# Autodesk Inventor assembly: 1103 Robot - Base2
(part 2 of 2)
- Mate:349: Flat Bearing Block:15 ↔ Nut 8-32 Nylock:9
- Mate:350: Screw 8-32 x 0.500''-Silver:13 ↔ Nut 8-32 Nylock:9
- Mate:351: Screw 8-32 x 0.500''-Silver:14 ↔ Nut 8-32 Nylock:8
- Mate:352: Flat Bearing Block:13 ↔ Nut 8-32 Nylock:10
- Mate:353: Flat Bearing Block:13 ↔ Nut 8-32 Nylock:11
- Mate:354: Screw 8-32 x 0.500''-Silver:9 ↔ Nut 8-32 Nylock:11
- Mate:355: Screw 8-32 x 0.500''-Silver:10 ↔ Nut 8-32 Nylock:10
- Mate:356: Flat Bearing Block:3 ↔ Nut 8-32 Nylock:12
- Mate:357: Flat Bearing Block:3 ↔ Nut 8-32 Nylock:13
- Mate:358: Flat Bearing Block:4 ↔ Nut 8-32 Nylock:14
- Mate:359: Flat Bearing Block:4 ↔ Nut 8-32 Nylock:15
- Mate:360: Flat Bearing Block:5 ↔ Nut 8-32 Nylock:17
- Mate:361: Flat Bearing Block:5 ↔ Nut 8-32 Nylock:16
- Mate:362: Screw 8-32 x 0.500''-Silver:6 ↔ Nut 8-32 Nylock:17
- Mate:363: Screw 8-32 x 0.500''-Silver:5 ↔ Nut 8-32 Nylock:16
- Mate:364: Screw 8-32 x 0.500''-Silver:4 ↔ Nut 8-32 Nylock:14
- Mate:365: Screw 8-32 x 0.500''-Silver:3 ↔ Nut 8-32 Nylock:15
- Mate:366: Screw 8-32 x 0.500''-Silver:1 ↔ Nut 8-32 Nylock:12
- Mate:367: Screw 8-32 x 0.500''-Silver:2 ↔ Nut 8-32 Nylock:13
- Mate:368: 2 x 6:1 ↔ Screw 8-32 x 0.250''-Silver:1
- Mate:369: 2 x 6:1 ↔ Screw 8-32 x 0.250''-Silver:2
- Mate:370: 2 x 6:2 ↔ Screw 8-32 x 0.250''-Silver:4
- Mate:371: 2 x 6:2 ↔ Screw 8-32 x 0.250''-Silver:3
- Mate:372: Standoff 0.50'':5 ↔ Screw 8-32 x 0.250''-Silver:1
- Mate:373: Standoff 0.50'':8 ↔ Screw 8-32 x 0.250''-Silver:2
- Mate:374: Standoff 0.50'':6 ↔ Screw 8-32 x 0.250''-Silver:4
- Mate:375: Standoff 0.50'':7 ↔ Screw 8-32 x 0.250''-Silver:3
- Mate:376: 2 x 6:4 ↔ Screw 8-32 x 0.250''-Silver:8
- Mate:377: 2 x 6:4 ↔ Screw 8-32 x 0.250''-Silver:7
- Mate:378: 2 x 6:3 ↔ Screw 8-32 x 0.250''-Silver:6
- Mate:379: 2 x 6:3 ↔ Screw 8-32 x 0.250''-Silver:5
- Mate:380: Standoff 0.50'':3 ↔ Screw 8-32 x 0.250''-Silver:6
- Mate:381: Standoff 0.50'':1 ↔ Screw 8-32 x 0.250''-Silver:5
- Mate:382: Standoff 0.50'':4 ↔ Screw 8-32 x 0.250''-Silver:7
- Mate:383: Standoff 0.50'':2 ↔ Screw 8-32 x 0.250''-Silver:8
- Mate:384: 4 Slotted Angle:1 ↔ Screw 8-32 x 0.250''-Silver:9
- Mate:385: 4 Slotted Angle:1 ↔ Screw 8-32 x 0.250''-Silver:10
- Mate:386: Standoff 0.50'':9 ↔ Screw 8-32 x 0.250''-Silver:9
- Mate:387: Standoff 0.50'':10 ↔ Screw 8-32 x 0.250''-Silver:10
- Mate:388: 4 Slotted Angle:2 ↔ Screw 8-32 x 0.250''-Silver:11
- Mate:389: 4 Slotted Angle:2 ↔ Screw 8-32 x 0.250''-Silver:12
- Mate:390: Standoff 0.50'':11 ↔ Screw 8-32 x 0.250''-Silver:12
- Mate:391: Standoff 0.50'':12 ↔ Screw 8-32 x 0.250''-Silver:11
- [Mate]: 4 x 6 cut:1 ↔ Screw 8-32 x 0.375''-Silver:1
- [Mate]: 4 x 6 cut:1 ↔ Screw 8-32 x 0.375''-Silver:2
- [Tangent] (0.2286 mm): 4 x 6 cut:1 ↔ Screw 8-32 x 0.375''-Silver:1
- [Tangent] (0.2286 mm): 4 x 6 cut:1 ↔ Screw 8-32 x 0.375''-Silver:1
- [Tangent] (0.2286 mm): 4 x 6 cut:1 ↔ Screw 8-32 x 0.375''-Silver:2
- [Tangent] (0.2286 mm): 4 x 6 cut:1 ↔ Screw 8-32 x 0.375''-Silver:2
- [Mate]: Ultrasonic Range Finder (Sensor):1 ↔ Nut 8-32 Keps:2
- [Mate]: Ultrasonic Range Finder (Sensor):1 ↔ Nut 8-32 Keps:1
- [Mate]: Screw 8-32 x 0.375''-Silver:1 ↔ Nut 8-32 Keps:1
- [Mate]: Screw 8-32 x 0.375''-Silver:2 ↔ Nut 8-32 Keps:2
- [Tangent] (0.2286 mm): 4 x 6 cut:2 ↔ Screw 8-32 x 0.375''-Silver:3
- [Tangent] (0.2286 mm): 4 x 6 cut:2 ↔ Screw 8-32 x 0.375''-Silver:3
- [Mate]: 4 x 6 cut:2 ↔ Screw 8-32 x 0.375''-Silver:3
- [Tangent] (0.2286 mm): 4 x 6 cut:2 ↔ Screw 8-32 x 0.375''-Silver:4
- [Tangent] (0.2286 mm): 4 x 6 cut:2 ↔ Screw 8-32 x 0.375''-Silver:4
- [Mate]: 4 x 6 cut:2 ↔ Screw 8-32 x 0.375''-Silver:4
- [Mate]: Ultrasonic Range Finder (Sensor):2 ↔ Nut 8-32 Keps:3
- [Mate]: Ultrasonic Range Finder (Sensor):2 ↔ Nut 8-32 Keps:4
- [Mate]: Nut 8-32 Keps:4 ↔ Screw 8-32 x 0.375''-Silver:3
- [Mate]: Nut 8-32 Keps:3 ↔ Screw 8-32 x 0.375''-Silver:4
- Mate:406: 4 x 6 cut:2 ↔ Screw 8-32 x 0.750''-Silver:1
- Mate:407: 4 x 6 cut:2 ↔ Screw 8-32 x 0.750''-Silver:2
- Mate:408: Spacer (Nylon), 0.375'':3 ↔ Screw 8-32 x 0.750''-Silver:1
- Mate:409: Spacer (Nylon), 0.375'':4 ↔ Screw 8-32 x 0.750''-Silver:2
- Mate:410: 4 Slotted Angle:2 ↔ Nut 8-32 Nylock:18
- Mate:411: 4 Slotted Angle:2 ↔ Nut 8-32 Nylock:19
- Mate:412: Screw 8-32 x 0.750''-Silver:2 ↔ Nut 8-32 Nylock:19
- Mate:413: Screw 8-32 x 0.750''-Silver:1 ↔ Nut 8-32 Nylock:18
- Mate:414: 4 x 6 cut:1 ↔ Screw 8-32 x 0.750''-Silver:3
- Mate:415: 4 x 6 cut:1 ↔ Screw 8-32 x 0.750''-Silver:4
- Mate:416: Spacer (Nylon), 0.375'':1 ↔ Screw 8-32 x 0.750''-Silver:3
- Mate:417: Spacer (Nylon), 0.375'':2 ↔ Screw 8-32 x 0.750''-Silver:4
- Mate:418: 4 Slotted Angle:1 ↔ Nut 8-32 Nylock:20
- Mate:419: 4 Slotted Angle:1 ↔ Nut 8-32 Nylock:21
- Mate:420: Screw 8-32 x 0.750''-Silver:4 ↔ Nut 8-32 Nylock:21
- Mate:421: Screw 8-32 x 0.750''-Silver:3 ↔ Nut 8-32 Nylock:20
- Tangent:171 (0.2311 mm): 1103 Custom Chassis:1 ↔ .375'' Screw & Nylock Nut:1
- Tangent:172 (0.2286 mm): 1103 Custom Chassis:1 ↔ .375'' Screw & Nylock Nut:1
- Mate:422: 5 x 24:1 ↔ .375'' Screw & Nylock Nut:1
- Mate:423: 1103 Custom Chassis:1 ↔ .375'' Screw & Nylock Nut:3
- Tangent:173 (0.2286 mm): 1103 Custom Chassis:1 ↔ .375'' Screw & Nylock Nut:3
- Tangent:174 (0.2286 mm): 1103 Custom Chassis:1 ↔ .375'' Screw & Nylock Nut:3
- Mate:424: 1103 Custom Chassis:1 ↔ .375'' Screw & Nylock Nut:4
- Mate:425: 1103 Custom Chassis:1 ↔ .375'' Screw & Nylock Nut:2
- Tangent:175 (0.2286 mm): 1103 Custom Chassis:1 ↔ .375'' Screw & Nylock Nut:2
- Tangent:176 (0.2286 mm): 1103 Custom Chassis:1 ↔ .375'' Screw & Nylock Nut:2
- Tangent:177: 1103 Custom Chassis:1 ↔ .375'' Screw & Nylock Nut:4
- Mate:426: 1103 Custom Chassis:1 ↔ .375'' Screw & Nylock Nut:5
- Mate:427: 1103 Custom Chassis:1 ↔ .375'' Screw & Nylock Nut:6
- Tangent:178 (0.2286 mm): 1103 Custom Chassis:1 ↔ .375'' Screw & Nylock Nut:5
- Tangent:179 (0.2286 mm): 1103 Custom Chassis:1 ↔ .375'' Screw & Nylock Nut:5
- Tangent:180 (0.2286 mm): 1103 Custom Chassis:1 ↔ .375'' Screw & Nylock Nut:6
- Tangent:181 (0.2286 mm): 1103 Custom Chassis:1 ↔ .375'' Screw & Nylock Nut:6
- Mate:428: 1103 Custom Chassis:1 ↔ .375'' Screw & Nylock Nut:7
- Mate:429: 1103 Custom Chassis:1 ↔ .375'' Screw & Nylock Nut:8
- Tangent:182 (0.2286 mm): 1103 Custom Chassis:1 ↔ .375'' Screw & Nylock Nut:8
- Tangent:183 (0.2286 mm): 1103 Custom Chassis:1 ↔ .375'' Screw & Nylock Nut:8
- Tangent:184 (0.2286 mm): 1103 Custom Chassis:1 ↔ .375'' Screw & Nylock Nut:7
- Tangent:185 (0.2286 mm): 1103 Custom Chassis:1 ↔ .375'' Screw & Nylock Nut:7
- Mate:430: 5 x 25 Custom:1 ↔ .375'' Screw & Nylock Nut:9
- Tangent:186 (0.2286 mm): 5 x 24:1 ↔ .375'' Screw & Nylock Nut:9
- Tangent:187 (0.2286 mm): 5 x 25 Custom:1 ↔ .375'' Screw & Nylock Nut:9
- Mate:431: 5 x 25 Custom:1 ↔ .375'' Screw & Nylock Nut:10
- Tangent:188 (0.2286 mm): 5 x 25 Custom:1 ↔ .375'' Screw & Nylock Nut:10
- Tangent:189 (0.2286 mm): 5 x 25 Custom:1 ↔ .375'' Screw & Nylock Nut:10
- Mate:432: 5 x 24:1 ↔ .375'' Screw & Nylock Nut:11
- Tangent:190 (0.2286 mm): 5 x 24:1 ↔ .375'' Screw & Nylock Nut:11
- Tangent:191 (0.2286 mm): 5 x 24:1 ↔ .375'' Screw & Nylock Nut:11
- Mate:433: 5 x 24:2 ↔ .375'' Screw & Nylock Nut:12
- Tangent:192 (0.2286 mm): 5 x 24:2 ↔ .375'' Screw & Nylock Nut:12
- Tangent:193 (0.2286 mm): 5 x 24:2 ↔ .375'' Screw & Nylock Nut:12
- Mate:434 (3.175 mm): 2 x 25:1 ↔ VEX-HINGE-1 RevA_1:1
- Mate:435 (3.175 mm): 2 x 25:1 ↔ VEX-HINGE-1 RevA 4x:1
- Mate:436: VEX-HINGE-1 RevA 4x:1 ↔ VEX-HINGE-PIN 4x:1
- Mate:437: VEX-HINGE-1 RevA_1:1 ↔ VEX-HINGE-PIN_1:1
- Flush:60: VEX-HINGE-1 RevA_1:1 ↔ VEX-HINGE-PIN_1:1
- Flush:61: VEX-HINGE-1 RevA 4x:1 ↔ VEX-HINGE-PIN 4x:1
- Flush:62: 2 x 25:1 ↔ VEX-HINGE-1 RevA_1:1
- Flush:63: 2 x 25:1 ↔ VEX-HINGE-1 RevA_1:1
- Flush:64: 2 x 25:1 ↔ VEX-HINGE-1 RevA 4x:1
- Flush:65: 2 x 25:1 ↔ VEX-HINGE-1 RevA 4x:1
- Flush:66 (2.3114 mm): VEX-HINGE-1 RevA_1:1
- Mate:448: 2 x 25:1 ↔ .375'' Screw & Nylock Nut:18
- Mate:449: 2 x 25:1 ↔ .375'' Screw & Nylock Nut:19
- Tangent:199 (0.2286 mm): 2 x 25:1 ↔ .375'' Screw & Nylock Nut:18
- Tangent:200 (0.2286 mm): 2 x 25:1 ↔ .375'' Screw & Nylock Nut:18
- Tangent:201 (0.2286 mm): 2 x 25:1 ↔ .375'' Screw & Nylock Nut:19
- Tangent:202 (0.2286 mm): 2 x 25:1 ↔ .375'' Screw & Nylock Nut:19
- Mate:450: 2 x 25:1 ↔ .375'' Screw & Nylock Nut:20
- Mate:451: 2 x 25:1 ↔ .375'' Screw & Nylock Nut:21
- Tangent:203 (0.2286 mm): 2 x 25:1 ↔ .375'' Screw & Nylock Nut:20
- Tangent:204 (0.2286 mm): 2 x 25:1 ↔ .375'' Screw & Nylock Nut:20
- Tangent:205 (0.2286 mm): 2 x 25:1 ↔ .375'' Screw & Nylock Nut:21
- Tangent:206 (0.2286 mm): 2 x 25:1 ↔ .375'' Screw & Nylock Nut:21
- Mate:452: 5 x 24:1 ↔ 2 x 25:1
- Flush:67: 5 x 24:1 ↔ 2 x 25:1
- Tangent:207 (0.2286 mm): 1103 Custom Chassis:1 ↔ .375'' Screw & Nylock Nut:4
- Mate:453: 2 x 25:1 ↔ Spacer (Nylon), 0.125'':1
- Tangent:208: VEX-HINGE-1 RevA 4x:1 ↔ Spacer (Nylon), 0.125'':1
- Tangent:209: VEX-HINGE-1 RevA 4x:1 ↔ Spacer (Nylon), 0.125'':1
- Mate:454: Screw 8-32 x 0.500''-Silver:19 ↔ Spacer (Nylon), 0.125'':1
- Mate:455: VEX-HINGE-1 RevA 4x:1 ↔ Screw 8-32 x 0.500''-Silver:19
- Mate:456: 2 x 25:1 ↔ Spacer (Nylon), 0.125'':2
- Mate:457: 2 x 25:1 ↔ Spacer (Nylon), 0.125'':3
- Mate:458: 2 x 25:1 ↔ Spacer (Nylon), 0.125'':4
- Mate:459: 2 x 25:1 ↔ Spacer (Nylon), 0.125'':5
- Tangent:210: VEX-HINGE-1 RevA_1:1 ↔ Spacer (Nylon), 0.125'':5
- Tangent:211: VEX-HINGE-1 RevA_1:1 ↔ Spacer (Nylon), 0.125'':5
- Tangent:212 (-0.2286 mm): VEX-HINGE-1 RevA_1:1 ↔ Spacer (Nylon), 0.125'':4
- Tangent:213 (-0.2286 mm): VEX-HINGE-1 RevA_1:1 ↔ Spacer (Nylon), 0.125'':4
- Tangent:214 (-0.2286 mm): VEX-HINGE-1 RevA_1:1 ↔ Spacer (Nylon), 0.125'':3
- Tangent:215 (-0.2286 mm): VEX-HINGE-1 RevA_1:1 ↔ Spacer (Nylon), 0.125'':3
- Tangent:216 (-0.2286 mm): VEX-HINGE-1 RevA 4x:1 ↔ Spacer (Nylon), 0.125'':2
- Tangent:217 (-0.2286 mm): VEX-HINGE-1 RevA 4x:1 ↔ Spacer (Nylon), 0.125'':2
- Mate:460: Screw 8-32 x 0.500''-Silver:20 ↔ Spacer (Nylon), 0.125'':2
- Mate:461: Screw 8-32 x 0.500''-Silver:21 ↔ Spacer (Nylon), 0.125'':3
- Mate:462: Screw 8-32 x 0.500''-Silver:22 ↔ Spacer (Nylon), 0.125'':4
- Mate:463: Screw 8-32 x 0.500''-Silver:23 ↔ Spacer (Nylon), 0.125'':5
- Mate:464: VEX-HINGE-1 RevA_1:1 ↔ Screw 8-32 x 0.500''-Silver:23
- Mate:465: VEX-HINGE-1 RevA_1:1 ↔ Screw 8-32 x 0.500''-Silver:22
- Mate:466: VEX-HINGE-1 RevA_1:1 ↔ Screw 8-32 x 0.500''-Silver:21
- Mate:467: VEX-HINGE-1 RevA 4x:1 ↔ Screw 8-32 x 0.500''-Silver:20
- Mate:468: 2 x 25:1 ↔ Nut 8-32 Nylock:22
- Mate:469: 2 x 25:1 ↔ Nut 8-32 Nylock:23
- Mate:470: 2 x 25:1 ↔ Nut 8-32 Nylock:24
- Mate:471: 2 x 25:1 ↔ Nut 8-32 Nylock:25
- Mate:472: 2 x 25:1 ↔ Nut 8-32 Nylock:26
- Mate:473: Screw 8-32 x 0.500''-Silver:23 ↔ Nut 8-32 Nylock:22
- Mate:474: Screw 8-32 x 0.500''-Silver:22 ↔ Nut 8-32 Nylock:23
- Mate:475: Screw 8-32 x 0.500''-Silver:21 ↔ Nut 8-32 Nylock:24
- Mate:476: Screw 8-32 x 0.500''-Silver:20 ↔ Nut 8-32 Nylock:25
- Mate:477: Screw 8-32 x 0.500''-Silver:19 ↔ Nut 8-32 Nylock:26
- Mate:478: Flat Bearing Block:8 ↔ 2-Wire Motor 393-Without Wire:2
- Mate:479: Flat Bearing Block:8 ↔ Screw 6-32 x 0.500''-Silver:9
- Mate:480: 2-Wire Motor 393-Without Wire:2 ↔ Screw 6-32 x 0.500''-Silver:9
- Mate:481: 5 x 24:1 ↔ Screw 6-32 x 0.500''-Silver:9
- Mate:482: 5 x 24:1 ↔ Drivetrain Encoder:1
- Flush:68: 5 x 24:1 ↔ Drivetrain Encoder:1
- Mate:483: 5 x 25 Custom:1 ↔ Drivetrain Encoder:1
- Mate:484: Drivetrain Encoder:1 ↔ Bearing Block:5
- Mate:485: 5 x 24:1 ↔ Bearing Block:5
- Tangent:220 (0.1905 mm): 5 x 24:1 ↔ Bearing Block:5
- Mate:486: 5 x 24:2 ↔ Bearing Block:6
- Tangent:221 (0.1905 mm): 5 x 24:2 ↔ Bearing Block:6
- Tangent:222 (0.1905 mm): 5 x 24:2 ↔ Bearing Block:6
- Tangent:223 (0.1905 mm): 5 x 24:2 ↔ Bearing Block:6
- Mate:487: Drivetrain Encoder:2 ↔ Bearing Block:6
- Mate:488: 5 x 24:2 ↔ Drivetrain Encoder:2
- Mate:489: 5 x 25 Custom:1 ↔ Drivetrain Encoder:2
- Mate:503: Screw 8-32 x 0.375''-Silver:7 ↔ Nut 8-32 Nylock:28
- Mate:504: Screw 8-32 x 0.375''-Silver:6 ↔ Nut 8-32 Nylock:27
- Mate:505: Nut 8-32 Nylock:27 ↔ Custom1x4 Mount:1
- Mate:506: Nut 8-32 Nylock:28 ↔ Custom1x4 Mount:1
- Mate:507: Screw 8-32 x 0.375''-Silver:5 ↔ Standoff 0.50'':13
- Mate:508: Custom1x4 Mount:1 ↔ Standoff 0.50'':13
- Mate:509: Screw 8-32 x 0.250''-Silver:13 ↔ Standoff 0.50'':13
- Mate:510 (1.1684 mm): Screw 8-32 x 0.250''-Silver:13 ↔ Standoff 0.50'':13
- Mate:511: 5 x 25 Custom:1 ↔ Standoff 0.50'':13
- Mate:512: 5 x 25 Custom:1 ↔ Custom1x4 Mount:1
- Mate:514 (2.3114 mm): 5 x 24:2 ↔ Screw 8-32 x 0.250''-Silver:14
- Mate:515 (2.3114 mm): 5 x 24:2 ↔ Screw 8-32 x 0.250''-Silver:14
- Mate:516: 5 x 24:2 ↔ Screw 8-32 x 0.250''-Silver:14
- Mate:517: Screw 8-32 x 0.250''-Silver:14 ↔ Standoff 0.50'':14
- Mate:518 (1.1684 mm): 5 x 24:2 ↔ Standoff 0.50'':14
- Mate:521: Standoff 0.50'':14 ↔ Screw 8-32 x 0.375''-Silver:8
- Mate:523: 5 x 25 Custom:1 ↔ On-Off Switch:1
- Angle:2 (90 deg): 5 x 25 Custom:1 ↔ On-Off Switch:1
- Mate:525: 5 x 25 Custom:1 ↔ Input Potentiometer:1
- Mate:526: 5 x 25 Custom:1 ↔ Input Potentiometer:2
- Mate:527 (2.3114 mm): 5 x 25 Custom:1 ↔ Input Potentiometer:1
- Mate:528 (2.3114 mm): 5 x 25 Custom:1 ↔ Input Potentiometer:1
- Mate:529 (2.3114 mm): 5 x 25 Custom:1 ↔ Input Potentiometer:1
- Mate:530 (2.3114 mm): 5 x 25 Custom:1 ↔ Input Potentiometer:2
- Mate:531 (2.3114 mm): 5 x 25 Custom:1 ↔ Input Potentiometer:2
- Mate:532 (2.3114 mm): 5 x 25 Custom:1 ↔ Input Potentiometer:2
- Mate:535 (1.27 mm): 5 x 25 Custom:1 ↔ Regulator Body:1
- Mate:536: 5 x 25 Custom:1 ↔ Regulator Nut:1
- Mate:537: Regulator Body:1 ↔ Regulator Nut:1
- Angle:3 (200 deg): 5 x 25 Custom:1 ↔ Regulator Body:1
- Mate:538: 5 x 25 Custom:1 ↔ Regulator Body:1
- Mate:539: 5 x 25 Custom:1 ↔ Tire Pump Fitting:1
- Mate:540: 5 x 25 Custom:1 ↔ Tire Pump Fitting:1
- Mate:541: Tier Pump Fitting Nut:1 ↔ Tire Pump Fitting:1
- Mate:542: 5 x 25 Custom:1 ↔ Tier Pump Fitting Nut:1
- Mate:544: Regulator Body:1 ↔ Fitting for Cylinders:1
- Angle:4 (340 deg): 5 x 25 Custom:1 ↔ Tire Pump Fitting:1
- Flush:71: 5 x 25 Custom:1 ↔ Metal L (3x2) :1
- Mate:545: 5 x 25 Custom:1 ↔ Metal L (3x2) :1
- Flush:546: 5 x 25 Custom:1 ↔ Metal L (3x2) :1
- Mate:546: 5 x 25 Custom:1 ↔ Metal L (3x2) :2
- Flush:547: 5 x 25 Custom:1 ↔ Metal L (3x2) :2
- Flush:548: 5 x 25 Custom:1 ↔ Metal L (3x2) :2
- Mate:550 (2.3114 mm): Metal L (3x2) :2 ↔ .375'' Screw & Nylock Nut:24
- Mate:551 (2.3114 mm): 5 x 25 Custom:1 ↔ .375'' Screw & Nylock Nut:24
- Mate:552: Metal L (3x2) :2 ↔ .375'' Screw & Nylock Nut:24
- Mate:553 (2.3114 mm): 5 x 25 Custom:1 ↔ .375'' Screw & Nylock Nut:22
- Mate:554 (2.3114 mm): Metal L (3x2) :1 ↔ .375'' Screw & Nylock Nut:22
- Mate:555: Metal L (3x2) :1 ↔ .375'' Screw & Nylock Nut:22
- Mate:559: Metal L (3x2) :2 ↔ Pneumatic Cylinder Mount:1
- Flush:549: Metal L (3x2) :2 ↔ Pneumatic Cylinder Mount:1
- Flush:550: Metal L (3x2) :2 ↔ Pneumatic Cylinder Mount:1
- Mate:560: Metal L (3x2) :1 ↔ Pneumatic Cylinder Mount:2
- Flush:551: Metal L (3x2) :1 ↔ Pneumatic Cylinder Mount:2
- Flush:552: Metal L (3x2) :1 ↔ Pneumatic Cylinder Mount:2
- Mate:561 (2.3114 mm): Pneumatic Cylinder Mount:2 ↔ Screw 8-32 x 0.500''-Silver:27
- Mate:562 (2.3114 mm): Pneumatic Cylinder Mount:2 ↔ Screw 8-32 x 0.500''-Silver:27
- [Mate] (2.3114 mm): Pneumatic Cylinder Mount:2 ↔ Screw 8-32 x 0.375''-Silver:9
- [Mate] (2.3114 mm): Pneumatic Cylinder Mount:2 ↔ Screw 8-32 x 0.375''-Silver:9
- [Mate]: Pneumatic Cylinder Mount:2 ↔ Screw 8-32 x 0.375''-Silver:9
- Mate:566: Pneumatic Cylinder Mount:2 ↔ Screw 8-32 x 0.500''-Silver:27
- Mate:567 (2.3114 mm): Pneumatic Cylinder Mount:1 ↔ Screw 8-32 x 0.500''-Silver:25
- Mate:568 (2.3114 mm): Pneumatic Cylinder Mount:1 ↔ Screw 8-32 x 0.500''-Silver:25
- Mate:569 (2.3114 mm): Pneumatic Cylinder Mount:1 ↔ Screw 8-32 x 0.375''-Silver:10
- Mate:570 (2.3114 mm): Pneumatic Cylinder Mount:1 ↔ Screw 8-32 x 0.375''-Silver:10
- Mate:571: Pneumatic Cylinder Mount:1 ↔ Screw 8-32 x 0.500''-Silver:25
- Mate:572: Pneumatic Cylinder Mount:1 ↔ Screw 8-32 x 0.375''-Silver:10
- Mate:573: Metal L (3x2) :1 ↔ Nut 8-32 Nylock:29
- Mate:574: 5 x 25 Custom:1 ↔ Nut 8-32 Nylock:30
- Mate:575: Metal L (3x2) :2 ↔ Nut 8-32 Nylock:31
- Mate:576: 5 x 25 Custom:1 ↔ Nut 8-32 Nylock:32
- Mate:577: Screw 8-32 x 0.375''-Silver:10 ↔ Nut 8-32 Nylock:31
- Mate:578: Screw 8-32 x 0.500''-Silver:25 ↔ Nut 8-32 Nylock:32
- Mate:579: Screw 8-32 x 0.375''-Silver:9 ↔ Nut 8-32 Nylock:29
- Mate:580: Screw 8-32 x 0.500''-Silver:27 ↔ Nut 8-32 Nylock:30
- Mate:581: 5 x 25:4 ↔ 1103 ID Plate (with hardware):1
- Mate:582: 5 x 25:4 ↔ 1103 ID Plate (with hardware):1
- Angle:5 (0 deg): 5 x 25:4 ↔ 1103 ID Plate (with hardware):1
- Mate:583: 5 x 25:2 ↔ 1103 ID Plate (with hardware):2
- Mate:584: 5 x 25:2 ↔ 1103 ID Plate (with hardware):2
- Angle:6 (0 deg): 5 x 25:2 ↔ 1103 ID Plate (with hardware):2
- Mate:585: 5 x 25:4 ↔ Plate 6x3:1
- Flush:553: 5 x 24:2 ↔ Plate 6x3:1
- Flush:554: 5 x 24:2 ↔ Plate 6x3:1
- Mate:586 (2.3114 mm): Plate 6x3:1 ↔ .375'' Screw & Nylock Nut:25
- Mate:587 (2.3114 mm): Plate 6x3:1 ↔ .375'' Screw & Nylock Nut:25
- Mate:588: Plate 6x3:1 ↔ .375'' Screw & Nylock Nut:25
- Mate:589 (2.3114 mm): Plate 6x3:1 ↔ .375'' Screw & Nylock Nut:26
- Mate:590 (2.3114 mm): Plate 6x3:1 ↔ .375'' Screw & Nylock Nut:26
- Mate:591: Plate 6x3:1 ↔ .375'' Screw & Nylock Nut:26
- Mate:592 (2.3114 mm): Plate 6x3:1 ↔ .375'' Screw & Nylock Nut:28
- Mate:593 (2.3114 mm): Plate 6x3:1 ↔ .375'' Screw & Nylock Nut:28
- Mate:594: Plate 6x3:1 ↔ .375'' Screw & Nylock Nut:28
- Mate:595 (2.3114 mm): Plate 6x3:1 ↔ .375'' Screw & Nylock Nut:27
- Mate:596 (2.3114 mm): 5 x 24:2 ↔ .375'' Screw & Nylock Nut:27
- Mate:597: Plate 6x3:1 ↔ .375'' Screw & Nylock Nut:27
- Mate:598: 5 x 24:1 ↔ Plate 6x3:2
- Flush:555: 5 x 24:1 ↔ Plate 6x3:2
- Flush:556: 5 x 24:1 ↔ Plate 6x3:2
- Mate:599 (2.3114 mm): 5 x 25:2 ↔ .375'' Screw & Nylock Nut:29
- Mate:600 (2.3114 mm): 5 x 25:2 ↔ .375'' Screw & Nylock Nut:29
- Mate:601: Plate 6x3:2 ↔ .375'' Screw & Nylock Nut:29
- Mate:602 (2.3114 mm): Plate 6x3:2 ↔ .375'' Screw & Nylock Nut:30
- Mate:603 (2.3114 mm): Plate 6x3:2 ↔ .375'' Screw & Nylock Nut:30
- Mate:604: Plate 6x3:2 ↔ .375'' Screw & Nylock Nut:30
- Mate:605 (2.3114 mm): Plate 6x3:2 ↔ .375'' Screw & Nylock Nut:32
- Mate:606 (2.3114 mm): Plate 6x3:2 ↔ .375'' Screw & Nylock Nut:32
- Mate:607: Plate 6x3:2 ↔ .375'' Screw & Nylock Nut:32
- Mate:608 (2.3114 mm): Plate 6x3:2 ↔ .375'' Screw & Nylock Nut:31
- Mate:609 (2.3114 mm): Plate 6x3:2 ↔ .375'' Screw & Nylock Nut:31
- Mate:610: Plate 6x3:2 ↔ .375'' Screw & Nylock Nut:31
- Mate:611: 1103 Custom Chassis:1 ↔ Aluminum L-Channel 1x5x2:1
- Flush:557: 1103 Custom Chassis:1 ↔ Aluminum L-Channel 1x5x2:1
- Flush:558: 1103 Custom Chassis:1 ↔ Aluminum L-Channel 1x5x2:1
- Mate:612: 1103 Custom Chassis:1 ↔ Aluminum L-Channel 1x5x2:2
- Flush:559: 1103 Custom Chassis:1 ↔ Aluminum L-Channel 1x5x2:2
- Flush:560: 1103 Custom Chassis:1 ↔ Aluminum L-Channel 1x5x2:2
- Mate:613 (2.3114 mm): 1103 Custom Chassis:1 ↔ .375'' Screw & Nylock Nut:33
- Mate:614 (2.3114 mm): 1103 Custom Chassis:1 ↔ .375'' Screw & Nylock Nut:33
- Mate:615: 1103 Custom Chassis:1 ↔ .375'' Screw & Nylock Nut:33
- Mate:616 (2.3114 mm): 1103 Custom Chassis:1 ↔ .375'' Screw & Nylock Nut:34
- Mate:617 (2.3114 mm): 1103 Custom Chassis:1 ↔ .375'' Screw & Nylock Nut:34
- Mate:618: 1103 Custom Chassis:1 ↔ .375'' Screw & Nylock Nut:34
- Mate:619 (2.3114 mm): 1103 Custom Chassis:1 ↔ .375'' Screw & Nylock Nut:35
- Mate:620 (2.3114 mm): Aluminum L-Channel 1x5x2:2 ↔ .375'' Screw & Nylock Nut:35
- Mate:621: 1103 Custom Chassis:1 ↔ .375'' Screw & Nylock Nut:35
- Mate:622 (2.3114 mm): 1103 Custom Chassis:1 ↔ .375'' Screw & Nylock Nut:36
- Mate:623 (2.3114 mm): 1103 Custom Chassis:1 ↔ .375'' Screw & Nylock Nut:36
- Mate:624: 1103 Custom Chassis:1 ↔ .375'' Screw & Nylock Nut:36
- Flush:561: Aluminum L-Channel 1x5x2:1 ↔ Plate 4x3:1
- Mate:625: Aluminum L-Channel 1x5x2:1 ↔ Plate 4x3:1
- Flush:562: Aluminum L-Channel 1x5x2:1 ↔ Plate 4x3:1
- Mate:626: Aluminum L-Channel 1x5x2:2 ↔ Plate 4x3:2
- Flush:627: Aluminum L-Channel 1x5x2:2 ↔ Plate 4x3:2
- Flush:628: Aluminum L-Channel 1x5x2:2 ↔ Plate 4x3:2
- Mate:627: Plate 4x3:1 ↔ Angle 2x2x10:1
- Flush:629: Plate 4x3:1 ↔ Angle 2x2x10:1
- Flush:630: Plate 4x3:1 ↔ Angle 2x2x10:1
- Mate:628: Plate 4x3:1 ↔ Angle 2x2x10:2
- Flush:631: Plate 4x3:1 ↔ Angle 2x2x10:2
- Flush:632: Plate 4x3:1 ↔ Angle 2x2x10:2
- Mate:629: Plate 4x3:2 ↔ Angle 2x2x10:3
- Flush:633: Plate 4x3:2 ↔ Angle 2x2x10:3
- Flush:634: Plate 4x3:2 ↔ Angle 2x2x10:3
- Mate:630: Plate 4x3:2 ↔ Angle 2x2x10:4
- Flush:635: Plate 4x3:2 ↔ Angle 2x2x10:4
- Flush:636: Plate 4x3:2 ↔ Angle 2x2x10:4
- Mate:631 (2.3114 mm): Angle 2x2x10:1 ↔ .375'' Screw & Nylock Nut:37
- Mate:632 (2.3114 mm): Angle 2x2x10:1 ↔ .375'' Screw & Nylock Nut:37
- Mate:633: Angle 2x2x10:1 ↔ .375'' Screw & Nylock Nut:37
- Mate:634 (2.3114 mm): Angle 2x2x10:2 ↔ .375'' Screw & Nylock Nut:38
- Mate:635 (2.3114 mm): Angle 2x2x10:2 ↔ .375'' Screw & Nylock Nut:38
- Mate:636: Angle 2x2x10:2 ↔ .375'' Screw & Nylock Nut:38
- Mate:637 (2.3114 mm): Angle 2x2x10:3 ↔ .375'' Screw & Nylock Nut:39
- Mate:638 (2.3114 mm): Angle 2x2x10:3 ↔ .375'' Screw & Nylock Nut:39
- Mate:639: Angle 2x2x10:3 ↔ .375'' Screw & Nylock Nut:39
- Mate:640 (2.3114 mm): Angle 2x2x10:4 ↔ .375'' Screw & Nylock Nut:40
- Mate:641 (2.3114 mm): Plate 4x3:2 ↔ .375'' Screw & Nylock Nut:40
- Mate:642: Angle 2x2x10:4 ↔ .375'' Screw & Nylock Nut:40
- Mate:643 (2.3114 mm): Angle 2x2x10:2 ↔ .375'' Screw & Nylock Nut:42
- Mate:644 (2.3114 mm): Angle 2x2x10:2 ↔ .375'' Screw & Nylock Nut:42
- Mate:645: Angle 2x2x10:2 ↔ .375'' Screw & Nylock Nut:42
- Mate:646 (2.3114 mm): Angle 2x2x10:1 ↔ .375'' Screw & Nylock Nut:41
- Mate:647 (2.3114 mm): Angle 2x2x10:1 ↔ .375'' Screw & Nylock Nut:41
- Mate:648: Angle 2x2x10:1 ↔ .375'' Screw & Nylock Nut:41
- Mate:649 (2.3114 mm): Angle 2x2x10:3 ↔ .375'' Screw & Nylock Nut:44
- Mate:650 (2.3114 mm): Angle 2x2x10:3 ↔ .375'' Screw & Nylock Nut:44
- Mate:651: Angle 2x2x10:3 ↔ .375'' Screw & Nylock Nut:44
- Mate:652 (2.3114 mm): Angle 2x2x10:4 ↔ .375'' Screw & Nylock Nut:43
- Mate:653 (2.3114 mm): Angle 2x2x10:4 ↔ .375'' Screw & Nylock Nut:43
- Mate:654: Angle 2x2x10:4 ↔ .375'' Screw & Nylock Nut:43
- Mate:655: Angle 2x2x10:2 ↔ 7.2V (Robot Battery) NiMH 3000mAh:1
- Mate:656 (13.716 mm): Angle 2x2x10:1 ↔ 7.2V (Robot Battery) NiMH 3000mAh:1
- Mate:657: Angle 2x2x10:4 ↔ 7.2V (Robot Battery) NiMH 3000mAh:2
- Mate:658 (13.716 mm): Angle 2x2x10:4 ↔ 7.2V (Robot Battery) NiMH 3000mAh:2
- Flush:637 (-2.54 mm): Angle 2x2x10:1 ↔ 7.2V (Robot Battery) NiMH 3000mAh:1
- Flush:638 (-2.54 mm): Angle 2x2x10:4 ↔ 7.2V (Robot Battery) NiMH 3000mAh:2
- Mate:659 (2.3114 mm): Angle 2x2x10:1 ↔ Screw 8-32 x 0.375''-Silver:11
- Mate:660 (2.3114 mm): Angle 2x2x10:1 ↔ Screw 8-32 x 0.375''-Silver:11
- Mate:661: Angle 2x2x10:1 ↔ Screw 8-32 x 0.375''-Silver:11
- Mate:662 (2.3114 mm): Angle 2x2x10:1 ↔ Screw 8-32 x 0.375''-Silver:12
- Mate:663 (2.3114 mm): Plate 4x3:1 ↔ Screw 8-32 x 0.375''-Silver:12
- Mate:664: Angle 2x2x10:1 ↔ Screw 8-32 x 0.375''-Silver:12
- Mate:665: Screw 8-32 x 0.375''-Silver:12 ↔ Nut 8-32 Nylock:34
- Mate:666: Screw 8-32 x 0.375''-Silver:11 ↔ Nut 8-32 Nylock:33
- Mate:667: Aluminum L-Channel 1x5x2:1 ↔ Nut 8-32 Nylock:33
- Mate:668: Aluminum L-Channel 1x5x2:1 ↔ Nut 8-32 Nylock:34
- Mate:669 (2.3114 mm): Aluminum L-Channel 1x5x2:2 ↔ Screw 8-32 x 0.375''-Silver:14
- Mate:670 (2.3114 mm): Aluminum L-Channel 1x5x2:2 ↔ Screw 8-32 x 0.375''-Silver:14
- Mate:671: Angle 2x2x10:4 ↔ Screw 8-32 x 0.375''-Silver:14
- Mate:672 (2.3114 mm): Angle 2x2x10:4 ↔ Screw 8-32 x 0.375''-Silver:13
- Mate:673 (2.3114 mm): Angle 2x2x10:4 ↔ Screw 8-32 x 0.375''-Silver:13
- Mate:674: Angle 2x2x10:4 ↔ Screw 8-32 x 0.375''-Silver:13
- Mate:675: Nut 8-32 Nylock:35 ↔ Screw 8-32 x 0.375''-Silver:14
- Mate:676: Screw 8-32 x 0.375''-Silver:13 ↔ Nut 8-32 Nylock:36
- Mate:677: Aluminum L-Channel 1x5x2:2 ↔ Nut 8-32 Nylock:35
- Mate:678: Aluminum L-Channel 1x5x2:2 ↔ Nut 8-32 Nylock:36
- Mate:679: Line Follower Sensor (Line Tracker):4 ↔ Screw 8-32 x 0.375''-Silver:8
- Mate:680: Line Follower Sensor (Line Tracker):4 ↔ Standoff 0.50'':14
- Angle:7 (180 deg): 5 x 24:2 ↔ Line Follower Sensor (Line Tracker):4
- Mate:681: Screw 8-32 x 0.375''-Silver:5 ↔ Custom1x4 Mount:1
- Mate:682 (2.3114 mm): 5 x 25 Custom:1 ↔ Screw 8-32 x 0.250''-Silver:13
- Mate:683: Screw 8-32 x 0.375''-Silver:6 ↔ Nut 8-32 Nylock:27
- Mate:684 (2.3114 mm): Screw 8-32 x 0.375''-Silver:6 ↔ Custom1x4 Mount:1
- Mate:685 (2.3114 mm): Nut 8-32 Nylock:27 ↔ Custom1x4 Mount:1
- Mate:686: Screw 8-32 x 0.375''-Silver:6 ↔ Line Follower Sensor (Line Tracker):1
- Mate:687: Screw 8-32 x 0.375''-Silver:5 ↔ Line Follower Sensor (Line Tracker):3
- Mate:688: Screw 8-32 x 0.375''-Silver:7 ↔ Line Follower Sensor (Line Tracker):2
- Mate:689: Custom1x4 Mount:1 ↔ Line Follower Sensor (Line Tracker):2
- Mate:690 (2.3114 mm): Screw 8-32 x 0.375''-Silver:7 ↔ Custom1x4 Mount:1
- Mate:691 (2.3114 mm): Nut 8-32 Nylock:28 ↔ Custom1x4 Mount:1
- Mate:692: Custom1x4 Mount:1 ↔ Line Follower Sensor (Line Tracker):3
- Mate:693: Custom1x4 Mount:1 ↔ Line Follower Sensor (Line Tracker):1
- Angle:8 (0 deg): Line Follower Sensor (Line Tracker):1 ↔ Line Follower Sensor (Line Tracker):3
- Angle:9 (0 deg): Line Follower Sensor (Line Tracker):2 ↔ Line Follower Sensor (Line Tracker):3
- Angle:10 (180 deg): 5 x 25 Custom:1 ↔ Line Follower Sensor (Line Tracker):3
- Mate:694: Regulator Body:1 ↔ Fitting for Cylinders:1
- Mate:695 (2.3114 mm): 5 x 24:1 ↔ Flat Bearing Block:7
- Mate:696 (2.3114 mm): 5 x 24:1 ↔ Flat Bearing Block:7
- Mate:697 (2.3114 mm): 5 x 24:1 ↔ .5'' Screw & Nylock Nut:2
- Mate:698: Flat Bearing Block:1 ↔ Flat Bearing Block:7
- Mate:699 (2.3114 mm): 5 x 25:2 ↔ 2x .5'' Screw & Nylock Nut:1
- Mate:700: Flat Bearing Block:7 ↔ Flat Bearing Block:10
- Mate:701 (2.3114 mm): 5 x 24:1 ↔ Bearing Block:4
- Mate:702: Flat Bearing Block:8 ↔ 2-Wire Motor 393-Without Wire:2
- Mate:703 (2.3114 mm): 5 x 24:1 ↔ Screw 6-32 x 0.500''-Silver:2
- Mate:704 (2.3114 mm): 5 x 24:1 ↔ Screw 6-32 x 0.500''-Silver:2
- Mate:705 (2.3114 mm): 5 x 24:1 ↔ Screw 6-32 x 0.500''-Silver:9
- Mate:706 (2.3114 mm): 5 x 24:1 ↔ Screw 6-32 x 0.500''-Silver:9
- Mate:707: Screw 6-32 x 0.500''-Silver:2 ↔ 2-Wire Motor 393-Without Wire:2
- Mate:708 (2.3114 mm): 5 x 24:2 ↔ Screw 6-32 x 0.500''-Silver:7
- Mate:709 (2.3114 mm): 5 x 24:2 ↔ Screw 6-32 x 0.500''-Silver:7
- Mate:710 (2.3114 mm): 5 x 24:2 ↔ Screw 6-32 x 0.500''-Silver:8
- Mate:711 (2.3114 mm): 5 x 24:2 ↔ Screw 6-32 x 0.500''-Silver:8
- Mate:712: Flat Bearing Block:12 ↔ 2-Wire Motor 393-Without Wire:3
- Mate:713: Pneumatic Cylinder Mount:2 ↔ Washer, Delrin:1
- Mate:714: Pneumatic Cylinder Mount:2 ↔ Washer, Delrin:2
- Mate:715: Pneumatic Cylinder Mount:2 ↔ Washer, Delrin:1
- Mate:716: Washer, Delrin:1 ↔ Washer, Delrin:2
- Mate:717: Pneumatic Cylinder Mount:1 ↔ Washer, Delrin:4
- Mate:718: Pneumatic Cylinder Mount:1 ↔ Washer, Delrin:3
- Mate:719: Pneumatic Cylinder Mount:1 ↔ Washer, Delrin:3
- Mate:720: Washer, Delrin:3 ↔ Washer, Delrin:4
- Mate:721: Pneumatic Cylinder Mount:1 ↔ Screw 8-32 x 0.875''-Silver:1
- Mate:722: Pneumatic Cylinder Mount:1 ↔ Screw 8-32 x 0.875''-Silver:1
- Mate:723: Nut 8-32 Nylock:37 ↔ Screw 8-32 x 0.875''-Silver:1
- Mate:724: Pneumatic Cylinder Mount:1 ↔ Nut 8-32 Nylock:37
- Mate:725: Pneumatic Cylinder Mount:2 ↔ Screw 8-32 x 0.875''-Silver:2
- Mate:726: Nut 8-32 Nylock:38 ↔ Screw 8-32 x 0.875''-Silver:2
- Mate:727: Pneumatic Cylinder Mount:2 ↔ Nut 8-32 Nylock:38
- Mate:728: Pneumatic Cylinder Mount:2 ↔ Screw 8-32 x 0.875''-Silver:2
- Mate:729: Screw 8-32 x 0.375''-Silver:6 ↔ Line Follower Sensor (Line Tracker):1
- Mate:730: Screw 8-32 x 0.375''-Silver:7 ↔ Line Follower Sensor (Line Tracker):2
- Mate:731: Screw 8-32 x 0.375''-Silver:5 ↔ Line Follower Sensor (Line Tracker):2
- Mate:732 (2.54 mm): 5 x 25 Custom:1 ↔ On-Off Switch:1
